# Autodesk Inventor assembly: installedConfig
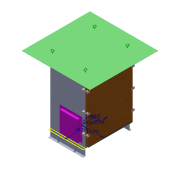
[picture p0: Inventor's stored thumbnail of the model, 180x180]
Saved by Autodesk Inventor 2017 (Build 210142000, 142)
## iProperties
Created: 2017-05-18
Part Number: installedConfig
Document SubType Name: Assembly
Designer: krosie
Author: krosie
## Documents named in this file (3)
- C:\Users\krosie\Google Drive\HERA\hera-cad\Node\Concept-ICTS\installedConfig.iam
- C:\Users\krosie\Google Drive\HERA\hera-cad\Node\protoPlinth.ipt
- C:\Users\krosie\Google Drive\HERA\hera-cad\Node\Concept-ICTS\ICTS-20170411\RD-A003-P000-REV0.iam
## Components (2 placed, 2 different names)
1. protoPlinth:1 — Mate:1, Tangent:1, Angle:1
2. RD-A003-P000-REV0:1 [sub-assembly] — Mate:1, Tangent:1, Angle:1
## Relationships (3: Mate 1, Tangent 1, Angle 1)
- Mate:1: protoPlinth:1 ↔ RD-A003-P000-REV0:1
- Tangent:1 (100 mm): protoPlinth:1 ↔ RD-A003-P000-REV0:1
- Angle:1 (0 deg): protoPlinth:1 ↔ RD-A003-P000-REV0:1
